# Autodesk Inventor assembly: Ensamblaje Uno
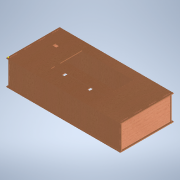
[picture p0: Inventor's stored thumbnail of the model, 180x180]
Saved by Autodesk Inventor 2020.3 (Build 243373000, 373)
## iProperties
Created: 2020-06-15
Part Number: Ensamblaje Uno
Document SubType Name: Assembly
Designer: miosh
Author: miosh
## Documents named in this file (5)
- D:\Archivos Carlos\Archivos Inventor\Ensamblaje Uno.iam
- D:\Archivos Carlos\Archivos Inventor\Frontal Arduino.ipt
- D:\Archivos Carlos\Archivos Inventor\Lado superior.ipt
- D:\Archivos Carlos\Archivos Inventor\Costados pequeños.ipt
- D:\Archivos Carlos\Archivos Inventor\Posterior Módulo Primario.ipt
## Components (6 placed, 4 different names)
1. Lado superior:1 — Coincidencia:3, Coincidencia:4, Nivelación:6, Coincidencia:5, Coincidencia:7, Coincidencia:8
2. Lado superior:2 — Nivelación:9, Coincidencia:9, Coincidencia:10, Coincidencia:12, Coincidencia:16
3. Frontal Arduino:1 — Coincidencia:3, Coincidencia:4, Nivelación:6, Coincidencia:6, Nivelación:9, Nivelación:10, Coincidencia:11
4. Costados pequeños:1 — Coincidencia:5, Coincidencia:6, Coincidencia:7, Coincidencia:8, Coincidencia:9, Coincidencia:10, Coincidencia:17
5. Costados pequeños:2 — Nivelación:10, Coincidencia:11, Coincidencia:12, Coincidencia:15
6. Posterior Módulo Primario:1 — Coincidencia:15, Coincidencia:16, Coincidencia:17
## Relationships (16: Mate 13, Flush 3)
- Coincidencia:3 [Mate]: Lado superior:1 ↔ Frontal Arduino:1
- Coincidencia:4 [Mate]: Lado superior:1 ↔ Frontal Arduino:1
- Nivelación:6 [Flush]: Lado superior:1 ↔ Frontal Arduino:1
- Coincidencia:5 [Mate]: Lado superior:1 ↔ Costados pequeños:1
- Coincidencia:6 [Mate]: Frontal Arduino:1 ↔ Costados pequeños:1
- Coincidencia:7 [Mate]: Lado superior:1 ↔ Costados pequeños:1
- Coincidencia:8 [Mate]: Lado superior:1 ↔ Costados pequeños:1
- Nivelación:9 [Flush]: Lado superior:2 ↔ Frontal Arduino:1
- Coincidencia:9 [Mate]: Lado superior:2 ↔ Costados pequeños:1
- Coincidencia:10 [Mate]: Lado superior:2 ↔ Costados pequeños:1
- Nivelación:10 [Flush]: Frontal Arduino:1 ↔ Costados pequeños:2
- Coincidencia:11 [Mate]: Frontal Arduino:1 ↔ Costados pequeños:2
- Coincidencia:12 [Mate]: Lado superior:2 ↔ Costados pequeños:2
- Coincidencia:15 [Mate]: Costados pequeños:2 ↔ Posterior Módulo Primario:1
- Coincidencia:16 [Mate]: Lado superior:2 ↔ Posterior Módulo Primario:1
- Coincidencia:17 [Mate]: Costados pequeños:1 ↔ Posterior Módulo Primario:1
